# Autodesk Inventor assembly: RailAttachmentAssembly
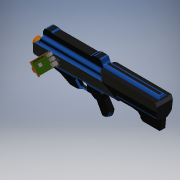
[picture p0: Inventor's stored thumbnail of the model, 180x180]
Saved by Autodesk Inventor 2018 (Build 220112000, 112)
## iProperties
Created: 2019-04-01
Part Number: RailAttachmentAssembly
Document SubType Name: Assembly
Designer: snipe
Author: snipe
## Documents named in this file (3)
- C:\Users\snipe\Documents\CPRE186-CAD\RailAttachmentAssemblyWithGun.iam
- C:\Users\snipe\Documents\CPRE186-CAD\RailAttachmentAssembly.iam
- C:\Users\snipe\Documents\CPRE186-CAD\NerfRivalZeus.ipt
## Components (2 placed, 2 different names)
1. RailAttachmentAssembly:1 [sub-assembly] — Mate:4
2. NerfRivalZeus:1 — Mate:2, Mate:1, Mate:3, Mate:4
## Relationships (4: Mate 4)
- Mate:2: NerfRivalZeus:1
- Mate:1: NerfRivalZeus:1
- Mate:3: NerfRivalZeus:1
- Mate:4: RailAttachmentAssembly:1 ↔ NerfRivalZeus:1
